# Autodesk Inventor assembly: 74. Комплект муфты со ступицей
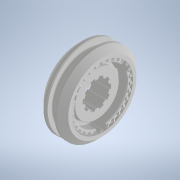
[picture p0: Inventor's stored thumbnail of the model, 180x180]
Saved by Autodesk Inventor 2021 (Build 250183000, 183)
## iProperties
Created: 2021-04-05
Part Number: 74. Комплект муфты со ступицей
Document SubType Name: Assembly
Designer: Данил
Author: Данил
## Documents named in this file (3)
- C:\Users\Данил\Desktop\Коробка передач\Детали\74. Комплект муфты со ступицей.iam
- C:\Users\Данил\Desktop\Коробка передач\Детали\74. Ступица муфты переключения третьей и четвертой передач.ipt
- C:\Users\Данил\Desktop\Коробка передач\Детали\72. Муфта синхронизатора.ipt
## Components (2 placed, 2 different names)
1. 74. Ступица муфты переключения третьей и четвертой передач:1 — Совмещение:1, Заподлицо:1, Угол:1
2. 72. Муфта синхронизатора:1 — Совмещение:1, Заподлицо:1, Угол:1
## Relationships (3: Mate 1, Flush 1, Angle 1)
- Совмещение:1 [Mate]: 74. Ступица муфты переключения третьей и четвертой передач:1 ↔ 72. Муфта синхронизатора:1
- Заподлицо:1 [Flush] (1.75 mm): 74. Ступица муфты переключения третьей и четвертой передач:1 ↔ 72. Муфта синхронизатора:1
- Угол:1 [Angle] (6 deg): 74. Ступица муфты переключения третьей и четвертой передач:1 ↔ 72. Муфта синхронизатора:1
